# Autodesk Inventor assembly: ElectronicsBatteryAssembly
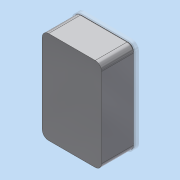
[picture p0: Inventor's stored thumbnail of the model, 180x180]
Saved by Autodesk Inventor 2017 (Build 210142000, 142)
## iProperties
Created: 2018-02-14
Part Number: ElectronicsBatteryAssembly
Document SubType Name: Assembly
Designer: Derek Wider
Author: Derek Wider
## Documents named in this file (6)
- G:\Projects\Submarine\Submarine-project\CAD\common\ElectronicsBatteryAssembly.iam
- G:\Projects\Submarine\Submarine-project\CAD\common\ElectronicsBatteryNoConnector.ipt
- G:\Projects\Submarine\Submarine-project\CAD\common\Connectors\XT60\XT60 Connector Female Connector.iam
- G:\Projects\Submarine\Submarine-project\CAD\fore\BatteryCaseSide1.ipt
- G:\Projects\Submarine\Submarine-project\CAD\fore\BatteryCaseSide2.ipt
- G:\Projects\Submarine\Submarine-project\CAD\fore\BatteryCaseORing.ipt
## Components (5 placed, 5 different names)
1. ElectronicsBatteryNoConnector:1 — Mate:1, Mate:2, Angle:1, Mate:3
2. XT60 Connector Female Connector:1 [sub-assembly] — Mate:1, Mate:2, Angle:1
3. BatteryCaseSide1:1 — Mate:3, Mate:4, Tangent:1, Tangent:2, Tangent:3, Tangent:4, Flush:1, Flush:2
4. BatteryCaseSide2:1 — Mate:4, Flush:1, Flush:2
5. BatteryCaseORing:1 — Tangent:1, Tangent:2, Tangent:3, Tangent:4
## Relationships (11: Mate 4, Tangent 4, Flush 2, Angle 1)
- Mate:1: ElectronicsBatteryNoConnector:1 ↔ XT60 Connector Female Connector:1
- Mate:2: ElectronicsBatteryNoConnector:1 ↔ XT60 Connector Female Connector:1
- Angle:1 (0 deg): ElectronicsBatteryNoConnector:1 ↔ XT60 Connector Female Connector:1
- Mate:3: ElectronicsBatteryNoConnector:1 ↔ BatteryCaseSide1:1
- Mate:4 (1.5875 mm): BatteryCaseSide1:1 ↔ BatteryCaseSide2:1
- Tangent:1: BatteryCaseSide1:1 ↔ BatteryCaseORing:1
- Tangent:2: BatteryCaseSide1:1 ↔ BatteryCaseORing:1
- Tangent:3 (0.9525 mm): BatteryCaseSide1:1 ↔ BatteryCaseORing:1
- Tangent:4 (0.9525 mm): BatteryCaseSide1:1 ↔ BatteryCaseORing:1
- Flush:1 (-1.27 mm): BatteryCaseSide1:1 ↔ BatteryCaseSide2:1
- Flush:2 (-1.27 mm): BatteryCaseSide1:1 ↔ BatteryCaseSide2:1
